# Autodesk Inventor assembly: Truss
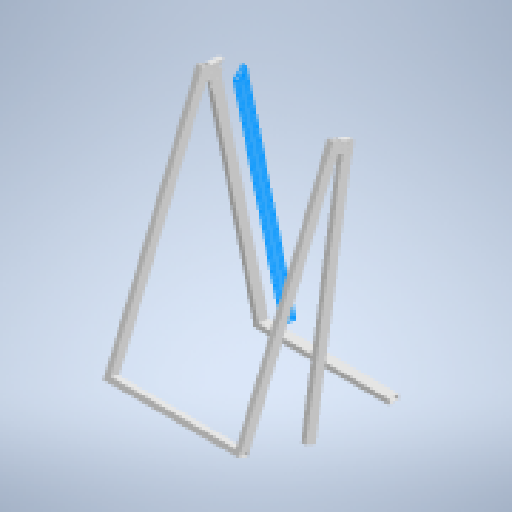
[picture p0: Inventor's stored thumbnail of the model, 512x512]
Saved by Autodesk Inventor 2023 (Build 270158000, 158)
## iProperties
Created: 2023-01-10
Part Number: Truss
Document SubType Name: Assembly
Designer: Terrence
Mass: 9567.53 g
Surface Area: 21493.6 cm^2
Volume: 3543.53 cm^3
Density: 2.7 g/cm^3
Author: Terrence
## Documents named in this file (6)
- C:\Users\Blank Slate\Documents\FRC 2023\Truss.iam
- C:\Users\Blank Slate\Documents\FRC 2023\Solid2_1.ipt
- C:\Users\Blank Slate\Documents\FRC 2023\Solid1_1.ipt
- C:\Users\Blank Slate\Documents\FRC 2023\Solid5.ipt
- C:\Users\Blank Slate\Documents\FRC 2023\Solid3_1.ipt
- C:\Users\Blank Slate\Documents\FRC 2023\Solid4.ipt
## Components (10 placed, 5 different names)
1. Solid3_1:1 — Flush:11, Mate:10, Flush:12, Flush:13, Mate:11, Flush:14
2. Solid4:5 — Mate:17, Mate:19, Mate:20
3. Solid4:4 — Insert:5, Insert:6
4. Solid2_1:2 — Insert:2, Flush:15, Mate:12, Mate:13, Mate:17, Mate:19
5. Solid1_1:2 — Mate:2, Flush:3, Flush:11, Mate:10, Flush:12, Mate:20
6. Solid5:2 — Mate:2, Flush:3, Insert:2
7. Solid2_1:3 — Insert:7, Insert:8
8. Solid1_1:3 — Flush:13, Mate:11, Flush:14, Insert:3, Insert:4
9. Solid5:3 — Insert:3, Insert:4, Insert:5, Insert:6, Insert:7, Insert:8
10. Solid3_1:2 — Flush:15, Mate:12, Mate:13
## Relationships (23: Mate 9, Flush 7, Insert 7)
- Mate:2: Solid1_1:2 ↔ Solid5:2
- Flush:3: Solid1_1:2 ↔ Solid5:2
- Insert:2: Solid2_1:2 ↔ Solid5:2
- Flush:11 (-171.45 mm): Solid3_1:1 ↔ Solid1_1:2
- Mate:10: Solid3_1:1 ↔ Solid1_1:2
- Flush:12: Solid3_1:1 ↔ Solid1_1:2
- Flush:13: Solid3_1:1 ↔ Solid1_1:3
- Mate:11: Solid3_1:1 ↔ Solid1_1:3
- Flush:14 (171.45 mm): Solid3_1:1 ↔ Solid1_1:3
- Flush:15 (-171.45 mm): Solid2_1:2 ↔ Solid3_1:2
- Mate:12: Solid2_1:2 ↔ Solid3_1:2
- Mate:13: Solid2_1:2 ↔ Solid3_1:2
- [Mate]: Solid4:5 ↔ Solid1_1:2
- [Flush]: Solid4:5 ↔ Solid2_1:2
- Mate:17: Solid4:5 ↔ Solid2_1:2
- Mate:19: Solid4:5 ↔ Solid2_1:2
- Mate:20: Solid4:5 ↔ Solid1_1:2
- Insert:3: Solid1_1:3 ↔ Solid5:3
- Insert:4: Solid1_1:3 ↔ Solid5:3
- Insert:5: Solid4:4 ↔ Solid5:3
- Insert:6: Solid4:4 ↔ Solid5:3
- Insert:7: Solid2_1:3 ↔ Solid5:3
- Insert:8: Solid2_1:3 ↔ Solid5:3
